# Autodesk Inventor assembly: Assembly3
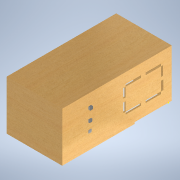
[picture p0: Inventor's stored thumbnail of the model, 180x180]
Saved by Autodesk Inventor 2022.2 (Build 262287000, 287)
## iProperties
Created: 2022-02-28
Part Number: Assembly3
Document SubType Name: Assembly
Designer: PRASHANTH
Author: PRASHANTH
## Documents named in this file (3)
- E:\BME\Autodesk Sample\Engg Exploration\Subsystem3-Button Unit\Assembly of Button Unit.iam
- E:\BME\Autodesk Sample\Engg Exploration\Subsystem3-Button Unit\button unit.ipt
- E:\BME\Autodesk Sample\Engg Exploration\Subsystem3-Button Unit\Buttons.ipt
## Components (4 placed, 2 different names)
1. button unit:1 — Mate:2
2. Buttons:1 — Mate:2, Flush:3
3. Buttons:2 — Flush:4
4. Buttons:3 — Flush:3, Flush:4
## Relationships (3: Flush 2, Mate 1)
- Mate:2: button unit:1 ↔ Buttons:1
- Flush:3: Buttons:1 ↔ Buttons:3
- Flush:4: Buttons:2 ↔ Buttons:3
